# Autodesk Inventor assembly: USB-C_PCB
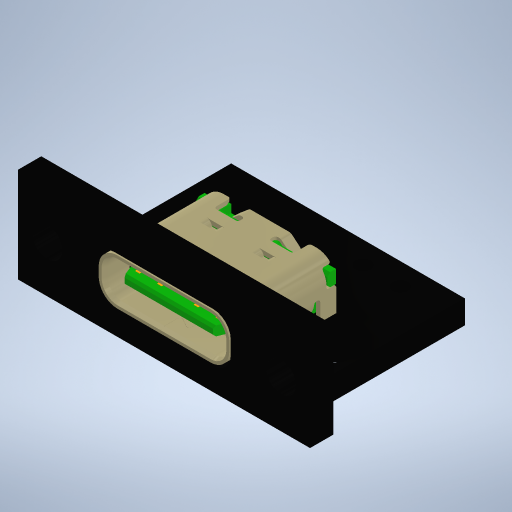
[picture p0: Inventor's stored thumbnail of the model, 512x512]
Saved by Autodesk Inventor 2024 (Build 280153000, 153)
## iProperties
Created: 2026-04-14
Part Number: USB-C_PCB
Document SubType Name: Assembly
Designer: Login
Author: Login
## Documents named in this file (4)
- D:\Inventor\Repositories\Temperature-Controller\Import\USB-C_PCB.iam
- D:\Inventor\Repositories\Temperature-Controller\Import\USB-C_face_plate.ipt
- D:\Inventor\Repositories\Temperature-Controller\Import\CONN-USB-C-DATA\CONN-USB-C-DATA.ipt
- D:\Inventor\Repositories\Temperature-Controller\Import\USB-C_BASE_plate.ipt
## Components (3 placed, 3 different names)
1. USB-C_face_plate:1 — Mate:1, Flush:1, Mate:2, Mate:4, Flush:2
2. CONN-USB-C-DATA:1 — Mate:1, Flush:1, Mate:2, Mate:3
3. USB-C_BASE_plate:1 — Mate:3, Mate:4, Flush:2
## Relationships (6: Mate 4, Flush 2)
- Mate:1 (0.1 mm): USB-C_face_plate:1 ↔ CONN-USB-C-DATA:1
- Flush:1: USB-C_face_plate:1 ↔ CONN-USB-C-DATA:1
- Mate:2 (0.1 mm): USB-C_face_plate:1 ↔ CONN-USB-C-DATA:1
- Mate:3: CONN-USB-C-DATA:1 ↔ USB-C_BASE_plate:1
- Mate:4: USB-C_face_plate:1 ↔ USB-C_BASE_plate:1
- Flush:2 (2 mm): USB-C_face_plate:1 ↔ USB-C_BASE_plate:1
